# Autodesk Inventor assembly: Assembly1
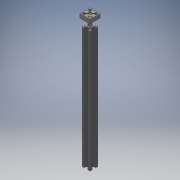
[picture p0: Inventor's stored thumbnail of the model, 180x180]
Saved by Autodesk Inventor 2019.4 (Build 234330000, 330)
## iProperties
Created: 2020-12-22
Part Number: Assembly1
Document SubType Name: Assembly
Designer: Jorian Brusind
Author: Jorian Brusind
## Documents named in this file (3)
- C:\Users\Jorian Brusind\Documents\GitHub\PersonalProjects\SpyderRobot\Inventor Files\Assembly1.iam
- C:\Users\Jorian Brusind\Documents\GitHub\PersonalProjects\SpyderRobot\Inventor Files\20 X 20 mm Extrusion 300mm.ipt
- C:\Users\Jorian Brusind\Documents\GitHub\PersonalProjects\SpyderRobot\Inventor Files\StepperMount.ipt
## Components (2 placed, 2 different names)
1. 20 X 20 mm Extrusion 300mm:1 — Flush:1, Flush:2
2. StepperMount:1 — Flush:1, Flush:2
## Relationships (2: Flush 2)
- Flush:1 (-2.5 mm): 20 X 20 mm Extrusion 300mm:1 ↔ StepperMount:1
- Flush:2 (-2.5 mm): 20 X 20 mm Extrusion 300mm:1 ↔ StepperMount:1
